# Autodesk Inventor assembly: Gripper
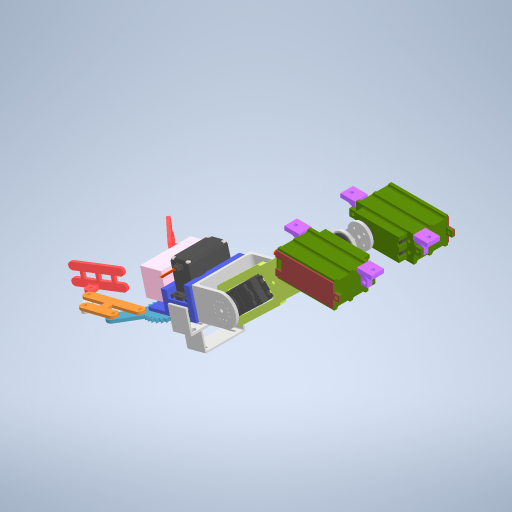
[picture p0: Inventor's stored thumbnail of the model, 512x512]
Saved by Autodesk Inventor 2023 (Build 270158000, 158)
## iProperties
Created: 2022-10-21
Part Number: Gripper
Document SubType Name: Assembly
Designer: amtat
Author: amtat
## Documents named in this file (21)
- C:\Users\matia\Downloads\Gripper\Gripper\Gripper.iam
- C:\Users\matia\Downloads\Gripper\Gripper\g1k.ipt
- C:\Users\matia\Downloads\Gripper\Gripper\TOWER PRO MG-995, ANALOG SERVO v9.iam
- C:\Users\matia\Downloads\Gripper\Gripper\dd3y.ipt
- C:\Users\matia\Downloads\Gripper\Gripper\antebrazo.ipt
- C:\Users\matia\Downloads\Gripper\Gripper\acople_1.ipt
- C:\Users\matia\Downloads\Gripper\Gripper\engranaje_acr.ipt
- C:\Users\matia\Downloads\Gripper\Gripper\acople_acr.ipt
- C:\Users\matia\Downloads\Gripper\Gripper\union_acr.ipt
- C:\Users\matia\Downloads\Gripper\Gripper\acople_gripper.ipt
- C:\Users\matia\Downloads\Gripper\Gripper\agarre_derecha.ipt
- C:\Users\matia\Downloads\Gripper\Gripper\agarre_izquierda.ipt
- C:\Users\matia\Downloads\Gripper\Gripper\acople_2.ipt
- C:\Users\matia\Downloads\Gripper\Gripper\soporte_sensor.ipt
- C:\Users\matia\Downloads\Gripper\Gripper\Ultra Sonic Sensor.ipt
- C:\Users\matia\Downloads\Gripper\Gripper\soporte_camara.ipt
- C:\Users\matia\Downloads\Gripper\Gripper\union_servos_1.ipt
- C:\Users\matia\Downloads\Gripper\Gripper\union_servos_2.ipt
- C:\Users\matia\Downloads\Gripper\Gripper\carcasa_servo.ipt
- C:\Users\matia\Downloads\Gripper\Gripper\tapa_carcasa.ipt
- C:\Users\matia\Downloads\Gripper\Gripper\base_servos.ipt
## Components (31 placed, 20 different names)
1. g1k:1 — Insert:1, Insert:2, Insert:9, Insert:10, Insert:12, Insert:13, Insert:28, Insert:29, Insert:42
2. TOWER PRO MG-995, ANALOG SERVO v9:1 [sub-assembly] — Insert:1, Insert:2, Insert:3, Insert:59
3. dd3y:1 — Insert:3, Insert:59
4. antebrazo:1 — Insert:4, Insert:5, Rotation:1, Insert:26, Insert:27, Insert:43, Insert:44, Insert:45, Insert:46
5. TOWER PRO MG-995, ANALOG SERVO v9:2 [sub-assembly] — Insert:4, Insert:5, Insert:8, Insert:11
6. acople_1:1 — Insert:8, Insert:9, Insert:10, Rotation:1, Insert:11
7. engranaje_acr:1 — Insert:12, Insert:14, Insert:15, Insert:19
8. engranaje_acr:2 — Insert:13, Insert:16, Insert:17, Insert:18
9. acople_acr:1 — Insert:14, Insert:15, Insert:21, Insert:23
10. acople_acr:2 — Insert:16, Insert:17, Insert:20, Insert:22
11. union_acr:1 — Insert:18, Insert:19
12. acople_gripper:1 — Insert:20, Insert:22, Insert:24
13. acople_gripper:2 — Insert:21, Insert:23, Insert:25
14. agarre_derecha:1 — Insert:24
15. agarre_izquierda:1 — Insert:25
16. acople_2:1 — Insert:26, Insert:27
17. soporte_sensor:1 — Insert:28, Insert:29, Mate:1, Mate:2, Flush:1
18. Ultra Sonic Sensor:1 — Mate:1, Mate:2, Flush:1
19. soporte_camara:1 — Insert:42
20. union_servos_1:1 — Insert:45, Insert:46, Insert:54
21. union_servos_2:1 — Insert:43, Insert:44, Insert:53
22. TOWER PRO MG-995, ANALOG SERVO v9:3 [sub-assembly] — Insert:47, Insert:48, Insert:54
23. carcasa_servo:1 — Insert:47, Insert:48, Insert:49, Flush:2, Flush:4, Insert:55, Mate:3, Insert:58, Mate:6
24. tapa_carcasa:1 — Insert:49, Flush:2
25. TOWER PRO MG-995, ANALOG SERVO v9:4 [sub-assembly] — Insert:53
26. carcasa_servo:2 — Flush:4, Insert:56, Mate:4, Insert:57, Mate:5
27. tapa_carcasa:2
28. base_servos:1 — Insert:56, Mate:4
29. base_servos:2 — Insert:55, Mate:3
30. base_servos:3 — Insert:57, Mate:5
31. base_servos:4 — Insert:58, Mate:6
## Relationships (56: Insert 45, Mate 6, Flush 4, RelateRotation 1)
- Insert:1: g1k:1 ↔ TOWER PRO MG-995, ANALOG SERVO v9:1
- Insert:2: g1k:1 ↔ TOWER PRO MG-995, ANALOG SERVO v9:1
- Insert:3: TOWER PRO MG-995, ANALOG SERVO v9:1 ↔ dd3y:1
- Insert:4: antebrazo:1 ↔ TOWER PRO MG-995, ANALOG SERVO v9:2
- Insert:5: antebrazo:1 ↔ TOWER PRO MG-995, ANALOG SERVO v9:2
- Insert:8: TOWER PRO MG-995, ANALOG SERVO v9:2 ↔ acople_1:1
- Insert:9: g1k:1 ↔ acople_1:1
- Insert:10: g1k:1 ↔ acople_1:1
- Rotation:1 [RelateRotation] (1 ul): antebrazo:1 ↔ acople_1:1
- Insert:11: TOWER PRO MG-995, ANALOG SERVO v9:2 ↔ acople_1:1
- Insert:12: g1k:1 ↔ engranaje_acr:1
- Insert:13: g1k:1 ↔ engranaje_acr:2
- Insert:14: engranaje_acr:1 ↔ acople_acr:1
- Insert:15: engranaje_acr:1 ↔ acople_acr:1
- Insert:16: engranaje_acr:2 ↔ acople_acr:2
- Insert:17: engranaje_acr:2 ↔ acople_acr:2
- Insert:18: engranaje_acr:2 ↔ union_acr:1
- Insert:19: engranaje_acr:1 ↔ union_acr:1
- Insert:20: acople_acr:2 ↔ acople_gripper:1
- Insert:21: acople_acr:1 ↔ acople_gripper:2
- Insert:22: acople_acr:2 ↔ acople_gripper:1
- Insert:23: acople_acr:1 ↔ acople_gripper:2
- Insert:24: acople_gripper:1 ↔ agarre_derecha:1
- Insert:25: acople_gripper:2 ↔ agarre_izquierda:1
- Insert:26: antebrazo:1 ↔ acople_2:1
- Insert:27: antebrazo:1 ↔ acople_2:1
- Insert:28: g1k:1 ↔ soporte_sensor:1
- Insert:29: g1k:1 ↔ soporte_sensor:1
- Mate:1 (0.15 mm): soporte_sensor:1 ↔ Ultra Sonic Sensor:1
- Mate:2 (1.75 mm): soporte_sensor:1 ↔ Ultra Sonic Sensor:1
- Flush:1 (2 mm): soporte_sensor:1 ↔ Ultra Sonic Sensor:1
- Insert:42: g1k:1 ↔ soporte_camara:1
- Insert:43: antebrazo:1 ↔ union_servos_2:1
- Insert:44: antebrazo:1 ↔ union_servos_2:1
- Insert:45: antebrazo:1 ↔ union_servos_1:1
- Insert:46: antebrazo:1 ↔ union_servos_1:1
- Insert:47: TOWER PRO MG-995, ANALOG SERVO v9:3 ↔ carcasa_servo:1
- Insert:48: TOWER PRO MG-995, ANALOG SERVO v9:3 ↔ carcasa_servo:1
- Insert:49: carcasa_servo:1 ↔ tapa_carcasa:1
- Flush:2: carcasa_servo:1 ↔ tapa_carcasa:1
- [Insert]: TOWER PRO MG-995, ANALOG SERVO v9:4 ↔ carcasa_servo:2
- [Insert]: TOWER PRO MG-995, ANALOG SERVO v9:4 ↔ carcasa_servo:2
- [Insert]: carcasa_servo:2 ↔ tapa_carcasa:2
- [Flush]: carcasa_servo:2 ↔ tapa_carcasa:2
- Insert:53: union_servos_2:1 ↔ TOWER PRO MG-995, ANALOG SERVO v9:4
- Insert:54: union_servos_1:1 ↔ TOWER PRO MG-995, ANALOG SERVO v9:3
- Flush:4: carcasa_servo:1 ↔ carcasa_servo:2
- Insert:55: carcasa_servo:1 ↔ base_servos:2
- Mate:3: carcasa_servo:1 ↔ base_servos:2
- Insert:56: carcasa_servo:2 ↔ base_servos:1
- Mate:4: carcasa_servo:2 ↔ base_servos:1
- Insert:57: carcasa_servo:2 ↔ base_servos:3
- Mate:5: carcasa_servo:2 ↔ base_servos:3
- Insert:58: carcasa_servo:1 ↔ base_servos:4
- Mate:6: carcasa_servo:1 ↔ base_servos:4
- Insert:59: TOWER PRO MG-995, ANALOG SERVO v9:1 ↔ dd3y:1
## Named parameters: d123_d119 = 0 mm, d124_d120 = 0 mm, d125_d121 = 0 mm, d126_d122 = 0 mm
